# Autodesk Inventor assembly: assembly
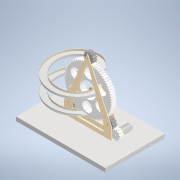
[picture p0: Inventor's stored thumbnail of the model, 180x180]
Saved by Autodesk Inventor 2021 (Build 250183000, 183)
## iProperties
Created: 2022-06-24
Part Number: assembly
Document SubType Name: Assembly
Designer: Suraj
Author: Suraj
## Documents named in this file (8)
- C:\Users\Suraj\Desktop\AUTODESK\Exploration\Run Machine.iam
- C:\Users\Suraj\Desktop\AUTODESK\Part1.ipt
- C:\Users\Suraj\Desktop\AUTODESK\CASE.ipt
- C:\Users\Suraj\Documents\Inventor\Content Center Files\R2021\en-US\Rivet GB_T 1011-1986\Rivet GB_T 1011-1986-4 X 30.ipt
- C:\Users\Suraj\Desktop\AUTODESK\Exploration\disk.ipt
- C:\Users\Suraj\Desktop\AUTODESK\Exploration\gear4.ipt
- C:\Users\Suraj\Desktop\AUTODESK\Exploration\base.ipt
- C:\Users\Suraj\Desktop\AUTODESK\Exploration\path.ipt
## Components (13 placed, 7 different names)
1. Part1:1 — Rotational:7
2. CASE:1 — Rigid:1
3. CASE:2 — Rigid:1, Rotational:1, Rotational:2, Rotational:3, Mate:2, Mate:5
4. Rivet GB/T 1011-1986 4 X 30:1 — Rotational:1, Rotational:5, Mate:4
5. Rivet GB/T 1011-1986 4 X 30:2 — Rotational:2, Rotational:4, Rotation:6
6. Rivet GB/T 1011-1986 4 X 30:3 — Rotational:3, Rotational:6, Rotation:2, Rotation:4, Rotation:6
7. disk:1 — Mate:1, Mate:3
8. gear4:1 — Rotational:6, Rotation:3
9. gear4:2 — Rotational:5
10. gear4:3 — Rotational:4
11. gear4:4 — Rotational:7, Flush:1, Mate:9, Mate:10, Rotation:3
12. base:1 — Flush:2, Mate:11, Mate:12
13. path:1 — Mate:13, Mate:14, Mate:15
## Relationships (26: Mate 12, RevoluteJoint 7, RelateRotation 4, Flush 2, WeldJoint 1)
- Rigid:1 [WeldJoint] (25 mm): CASE:1 ↔ CASE:2
- Rotational:1 [RevoluteJoint]: CASE:2 ↔ Rivet GB/T 1011-1986 4 X 30:1
- Rotational:2 [RevoluteJoint]: CASE:2 ↔ Rivet GB/T 1011-1986 4 X 30:2
- Rotational:3 [RevoluteJoint]: CASE:2 ↔ Rivet GB/T 1011-1986 4 X 30:3
- Rotational:6 [RevoluteJoint] (-5 mm): Rivet GB/T 1011-1986 4 X 30:3 ↔ gear4:1
- Rotational:4 [RevoluteJoint] (5 mm): Rivet GB/T 1011-1986 4 X 30:2 ↔ gear4:3
- Rotational:5 [RevoluteJoint] (5 mm): Rivet GB/T 1011-1986 4 X 30:1 ↔ gear4:2
- Mate:1 (-12.5 mm): disk:1
- Mate:2 (-15 mm): CASE:2
- Mate:3: disk:1
- Mate:4: Rivet GB/T 1011-1986 4 X 30:1
- Mate:5 (-160 mm): CASE:2
- Rotational:7 [RevoluteJoint] (13.5 mm): Part1:1 ↔ gear4:4
- Flush:1 (-10 mm): gear4:4
- Mate:9 (-130 mm): gear4:4
- Mate:10 (135 mm): gear4:4
- Rotation:2 [RelateRotation] (1 ul): Rivet GB/T 1011-1986 4 X 30:3
- Rotation:3 [RelateRotation] (1 ul): gear4:1 ↔ gear4:4
- Rotation:4 [RelateRotation] (1 ul): Rivet GB/T 1011-1986 4 X 30:3
- Rotation:6 [RelateRotation] (1 ul): Rivet GB/T 1011-1986 4 X 30:2 ↔ Rivet GB/T 1011-1986 4 X 30:3
- Flush:2 (160 mm): base:1
- Mate:11 (-150 mm): base:1
- Mate:12 (-225 mm): base:1
- Mate:13 (-15 mm): path:1
- Mate:14 (-15 mm): path:1
- Mate:15 (45.5 mm): path:1
